# Autodesk Inventor assembly: CM_Magnet_V2
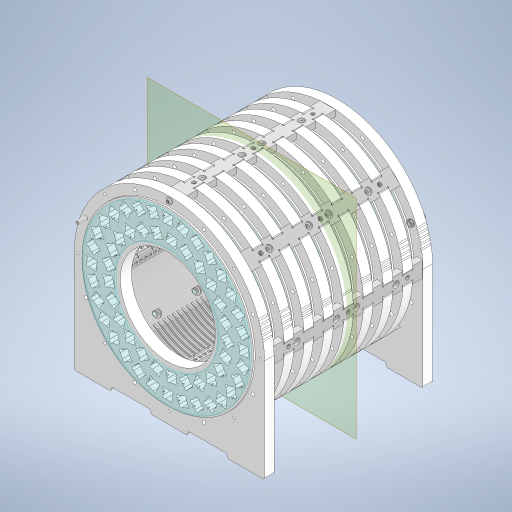
[picture p0: Inventor's stored thumbnail of the model, 512x512]
Saved by Autodesk Inventor 2024.3 (Build 283343000, 343)
## iProperties
Created: 2023-07-27
Part Number: CM_Magnet_V2
Document SubType Name: Assembly
Designer: Joshua Harper
Author: Joshua Harper
## Documents named in this file (15)
- G:\My Drive\OSI_Mini_CAD\OSII_MINI_V1_shared - Copy\CM_Magnet_V2.iam
- G:\My Drive\OSI_Mini_CAD\OSII_MINI_V1_shared - Copy\Ring_0.ipt
- G:\My Drive\OSI_Mini_CAD\OSII_MINI_V1_shared - Copy\Ring_1.ipt
- G:\My Drive\OSI_Mini_CAD\OSII_MINI_V1_shared - Copy\Ring_2.ipt
- G:\My Drive\OSI_Mini_CAD\OSII_MINI_V1_shared - Copy\Ring_3.ipt
- G:\My Drive\OSI_Mini_CAD\OSII_MINI_V1_shared - Copy\Ring_4.ipt
- G:\My Drive\OSI_Mini_CAD\OSII_MINI_V1_shared - Copy\M4_threaded_brass.ipt
- G:\My Drive\OSI_Mini_CAD\OSII_MINI_V1_shared - Copy\93187A150_NO THREADS_Brass Thin Hex Nut.ipt
- G:\My Drive\OSI_Mini_CAD\OSII_MINI_V1_shared - Copy\98691A114_General Purpose Brass Washer.ipt
- G:\My Drive\OSI_Mini_CAD\OSII_MINI_V1_shared - Copy\94500A283_NO THREADS_316 Stainless Steel Button Head Hex Drive Screws.ipt
- G:\My Drive\OSI_Mini_CAD\OSII_MINI_V1_shared - Copy\94500A283_NO THREADS_316 Stainless Steel Button Head Hex Drive Screws_MIR.ipt
- G:\My Drive\OSI_Mini_CAD\OSII_MINI_V1_shared - Copy\Lid_A.ipt
- G:\My Drive\OSI_Mini_CAD\OSII_MINI_V1_shared - Copy\Lid_B.ipt
- G:\My Drive\OSI_Mini_CAD\OSII_MINI_V1_shared - Copy\Locating_bar_V2.ipt
- G:\My Drive\OSI_Mini_CAD\OSII_MINI_V1_shared - Copy\Shim_Assem_V4.iam
## Components (34 placed, 14 different names)
1. Ring_0:1 — Mate:4, Mate:5, Mate:16, Mate:71, Flush:3, Flush:4, Flush:5, Flush:6, Flush:8, Flush:9, Flush:13
2. Ring_1:1 — Mate:5, Mate:17, Flush:3, Mate:84, Flush:9, Flush:10
3. Ring_1:2 — Mate:3, Mate:4, Mate:10, Mate:16, Flush:7, Flush:8
4. Ring_2:1 — Mate:6, Mate:17, Flush:4, Mate:86, Flush:10, Flush:11
5. Ring_2:2 — Mate:2, Mate:3, Mate:9, Mate:10, Mate:82, Flush:7, Flush:12, Mate:88
6. Ring_3:1 — Mate:6, Mate:7, Flush:5, Mate:85, Flush:11
7. Ring_3:2 — Mate:1, Mate:2, Mate:8, Mate:9, Flush:12
8. Ring_4:1 — Mate:7, Flush:6, Mate:72, Mate:73, Mate:74, Mate:79, Mate:80, Mate:81, Mate:84, Mate:85, Mate:86, Mate:87
9. Ring_4:2 — Mate:1, Mate:8, Mate:26, Mate:62, Mate:63, Mate:68, Mate:78
10. 98691A114_General Purpose Brass Washer:2 — Mate:63, Mate:66
11. 98691A114_General Purpose Brass Washer:1 — Mate:62, Mate:67
12. 93187A150_NO THREADS_Brass Thin Hex Nut:2 — Mate:66
13. 93187A150_NO THREADS_Brass Thin Hex Nut:1 — Mate:67
14. 94500A283_NO THREADS_316 Stainless Steel Button Head Hex Drive Screws:1 — Mate:68, Mate:78
15. 94500A283_NO THREADS_316 Stainless Steel Button Head Hex Drive Screws_MIR:1 — Mate:72, Mate:73, Mate:83
16. M4_threaded_brass:1 — Mate:26, Mate:74
17. Shim_Assem_V4:1 [sub-assembly] — Mate:87, Mate:88, Mate:89
18. Lid_B:1 — Mate:79, Mate:80
19. Lid_B:2
20. Lid_A:1 — Mate:71
21. Lid_A:2
22. Lid_A:3
23. Lid_A:4
24. Lid_A:5
25. Lid_A:6
26. Lid_A:7
27. Locating_bar_V2:1 — Mate:81, Mate:82, Mate:83
28. Locating_bar_V2:2
29. Locating_bar_V2:3
30. Locating_bar_V2:4
31. Locating_bar_V2:5
32. Locating_bar_V2:6
33. Locating_bar_V2:7
34. Locating_bar_V2:8 — Mate:89
## Component patterns: (2 elements, first: Lid_B:1), (7 elements, first: Lid_A:1), (8 elements, first: Locating_bar_V2:1)
## Relationships (45: Mate 34, Flush 11)
- Mate:1 (11 mm): Ring_3:2 ↔ Ring_4:2
- Mate:2 (11 mm): Ring_2:2 ↔ Ring_3:2
- Mate:3 (11 mm): Ring_1:2 ↔ Ring_2:2
- Mate:4 (11 mm): Ring_0:1 ↔ Ring_1:2
- Mate:5 (11 mm): Ring_0:1 ↔ Ring_1:1
- Mate:6 (11 mm): Ring_2:1 ↔ Ring_3:1
- Mate:7 (11 mm): Ring_3:1 ↔ Ring_4:1
- Mate:8: Ring_3:2 ↔ Ring_4:2
- Mate:9: Ring_2:2 ↔ Ring_3:2
- Mate:10: Ring_1:2 ↔ Ring_2:2
- Mate:16: Ring_0:1 ↔ Ring_1:2
- Mate:17 (11 mm): Ring_1:1 ↔ Ring_2:1
- Mate:26: Ring_4:2 ↔ M4_threaded_brass:1
- Mate:62: Ring_4:2 ↔ 98691A114_General Purpose Brass Washer:1
- Mate:63: Ring_4:2 ↔ 98691A114_General Purpose Brass Washer:2
- Mate:66: 98691A114_General Purpose Brass Washer:2 ↔ 93187A150_NO THREADS_Brass Thin Hex Nut:2
- Mate:67: 98691A114_General Purpose Brass Washer:1 ↔ 93187A150_NO THREADS_Brass Thin Hex Nut:1
- Mate:68: Ring_4:2 ↔ 94500A283_NO THREADS_316 Stainless Steel Button Head Hex Drive Screws:1
- Mate:71: Ring_0:1 ↔ Lid_A:1
- Flush:3: Ring_0:1 ↔ Ring_1:1
- Flush:4: Ring_0:1 ↔ Ring_2:1
- Flush:5: Ring_0:1 ↔ Ring_3:1
- Flush:6: Ring_0:1 ↔ Ring_4:1
- Mate:72: Ring_4:1 ↔ 94500A283_NO THREADS_316 Stainless Steel Button Head Hex Drive Screws_MIR:1
- Mate:73: Ring_4:1 ↔ 94500A283_NO THREADS_316 Stainless Steel Button Head Hex Drive Screws_MIR:1
- Mate:74: Ring_4:1 ↔ M4_threaded_brass:1
- Mate:78: Ring_4:2 ↔ 94500A283_NO THREADS_316 Stainless Steel Button Head Hex Drive Screws:1
- Mate:79: Ring_4:1 ↔ Lid_B:1
- Mate:80 (0.5 mm): Ring_4:1 ↔ Lid_B:1
- Mate:81: Ring_4:1 ↔ Locating_bar_V2:1
- Mate:82: Ring_2:2 ↔ Locating_bar_V2:1
- Mate:83: 94500A283_NO THREADS_316 Stainless Steel Button Head Hex Drive Screws_MIR:1 ↔ Locating_bar_V2:1
- Mate:84: Ring_1:1 ↔ Ring_4:1
- Mate:85: Ring_3:1 ↔ Ring_4:1
- Mate:86: Ring_2:1 ↔ Ring_4:1
- Flush:7: Ring_1:2 ↔ Ring_2:2
- Flush:8: Ring_0:1 ↔ Ring_1:2
- Flush:9: Ring_0:1 ↔ Ring_1:1
- Flush:10: Ring_1:1 ↔ Ring_2:1
- Flush:11: Ring_2:1 ↔ Ring_3:1
- Flush:12: Ring_2:2 ↔ Ring_3:2
- Flush:13 (-8 mm): Ring_0:1
- Mate:87: Ring_4:1 ↔ Shim_Assem_V4:1
- Mate:88: Ring_2:2 ↔ Shim_Assem_V4:1
- Mate:89: Shim_Assem_V4:1 ↔ Locating_bar_V2:8
## Named parameters: r_space = 11 mm
